# Autodesk Inventor assembly: LR_07
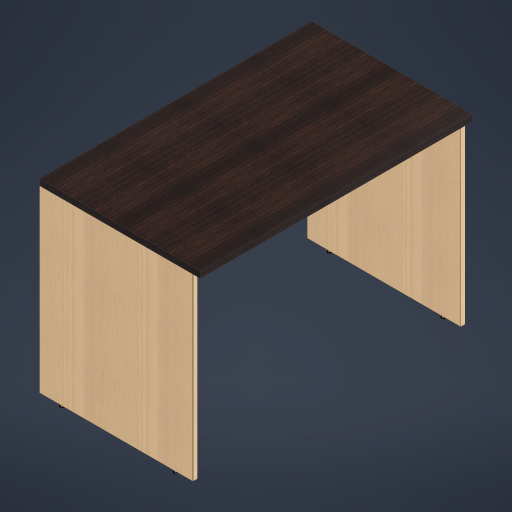
[picture p0: Inventor's stored thumbnail of the model, 512x512]
Saved by Autodesk Inventor 2024.3 (Build 283343000, 343)
## iProperties
Created: 2013-04-03
Part Number: LR_07
Document SubType Name: Assembly
Designer: User
Description: Table
Author: User
## Documents named in this file (10)
- C:\W4INV 2024 Design\PROJECTS\Living Room\Table\LR_07.iam
- C:\W4INV 2024 Design\PROJECTS\Samples\Living Room\Table\LR_0703.ipt
- C:\W4INV 2024 Design\PROJECTS\Samples\Living Room\Table\LR_0701.ipt
- C:\W4INV 2024 Design\PROJECTS\Samples\Living Room\Table\LR_0700.ipt
- C:\W4INV 2024 Design\PROJECTS\Samples\Living Room\Table\LR_0702.ipt
- C:\W4INV 2024 Design\_LIBRARY\Fixed joints\Minifix joint\MINIFIX D15 v2\Minifix D15 & Dowel L34 & Cap D15 PB T18 LH.ipt
- C:\W4INV 2024 Design\_LIBRARY\Fixed joints\Minifix joint\MINIFIX D15 v2\Minifix D15 & Dowel L34 & Cap D15 PB T18 RH.ipt
- C:\W4INV 2024 Design\_LIBRARY\Supports and legs\Supports\ADJUSTABLE SUPPORT\Support M6 H27 D18 with Bushing SB T18.ipt
- C:\W4INV 2023 Design\LIBRARY\Supports and legs\Supports\ADJUSTABLE SUPPORT.ipt
- C:\W4INV 2023 Design\LIBRARY\Fixed joints\Minifix joint\MINIFIX D15 v2.ipt
## Components (16 placed, 7 different names)
1. LR_0703-Desktop:1 — Mate:18, Mate:20, Mate:22, Mate:24
2. LR_0701-Left Leg:1 — Flush:1, Flush:2, Flush:25, Mate:10, Mate:12, Flush:27, Mate:14, Mate:16, Flush:29, Flush:31, Mate:26, Mate:30
3. LR_0700-Right Leg:1 — Flush:26, Flush:28, Flush:30, Flush:32, Mate:28, Mate:32
4. LR_0702-Support:1 — Flush:7, Flush:8, Flush:33, Flush:34, Flush:35, Flush:36
5. Support M6 H27 D18 with Bushing SB T18:5 — Mate:9, Flush:25, Mate:10
6. Support M6 H27 D18 with Bushing SB T18:6 — Mate:11, Flush:26, Mate:12
7. Support M6 H27 D18 with Bushing SB T18:7 — Mate:13, Flush:27, Mate:14
8. Support M6 H27 D18 with Bushing SB T18:8 — Mate:15, Flush:28, Mate:16
9. Minifix D15 & Dowel L34 & Cap D15 PB T18 LH:1 — Mate:17, Flush:29, Mate:18
10. Minifix D15 & Dowel L34 & Cap D15 PB T18 RH:2 — Mate:19, Flush:30, Mate:20
11. Minifix D15 & Dowel L34 & Cap D15 PB T18 RH:3 — Mate:21, Flush:31, Mate:22
12. Minifix D15 & Dowel L34 & Cap D15 PB T18 LH:4 — Mate:23, Flush:32, Mate:24
13. Minifix D15 & Dowel L34 & Cap D15 PB T18 LH:5 — Mate:25, Mate:26, Flush:33
14. Minifix D15 & Dowel L34 & Cap D15 PB T18 RH:6 — Mate:27, Mate:28, Flush:34
15. Minifix D15 & Dowel L34 & Cap D15 PB T18 RH:7 — Mate:29, Mate:30, Flush:35
16. Minifix D15 & Dowel L34 & Cap D15 PB T18 LH:8 — Mate:31, Mate:32, Flush:36
## Relationships (40: Mate 24, Flush 16)
- Flush:1 (-80 mm): LR_0701-Left Leg:1
- Flush:2 (-80 mm): LR_0701-Left Leg:1
- Flush:7 (-60 mm): LR_0702-Support:1
- Flush:8 (-60 mm): LR_0702-Support:1
- Mate:9: Support M6 H27 D18 with Bushing SB T18:5
- Flush:25 (9 mm): LR_0701-Left Leg:1 ↔ Support M6 H27 D18 with Bushing SB T18:5
- Mate:10 (17.5 mm): LR_0701-Left Leg:1 ↔ Support M6 H27 D18 with Bushing SB T18:5
- Mate:11: Support M6 H27 D18 with Bushing SB T18:6
- Flush:26 (9 mm): LR_0700-Right Leg:1 ↔ Support M6 H27 D18 with Bushing SB T18:6
- Mate:12 (17.5 mm): LR_0701-Left Leg:1 ↔ Support M6 H27 D18 with Bushing SB T18:6
- Mate:13: Support M6 H27 D18 with Bushing SB T18:7
- Flush:27 (9 mm): LR_0701-Left Leg:1 ↔ Support M6 H27 D18 with Bushing SB T18:7
- Mate:14 (17.5 mm): LR_0701-Left Leg:1 ↔ Support M6 H27 D18 with Bushing SB T18:7
- Mate:15: Support M6 H27 D18 with Bushing SB T18:8
- Flush:28 (9 mm): LR_0700-Right Leg:1 ↔ Support M6 H27 D18 with Bushing SB T18:8
- Mate:16 (17.5 mm): LR_0701-Left Leg:1 ↔ Support M6 H27 D18 with Bushing SB T18:8
- Mate:17: Minifix D15 & Dowel L34 & Cap D15 PB T18 LH:1
- Flush:29 (18 mm): LR_0701-Left Leg:1 ↔ Minifix D15 & Dowel L34 & Cap D15 PB T18 LH:1
- Mate:18: LR_0703-Desktop:1 ↔ Minifix D15 & Dowel L34 & Cap D15 PB T18 LH:1
- Mate:19: Minifix D15 & Dowel L34 & Cap D15 PB T18 RH:2
- Flush:30 (18 mm): LR_0700-Right Leg:1 ↔ Minifix D15 & Dowel L34 & Cap D15 PB T18 RH:2
- Mate:20: LR_0703-Desktop:1 ↔ Minifix D15 & Dowel L34 & Cap D15 PB T18 RH:2
- Mate:21: Minifix D15 & Dowel L34 & Cap D15 PB T18 RH:3
- Flush:31 (18 mm): LR_0701-Left Leg:1 ↔ Minifix D15 & Dowel L34 & Cap D15 PB T18 RH:3
- Mate:22: LR_0703-Desktop:1 ↔ Minifix D15 & Dowel L34 & Cap D15 PB T18 RH:3
- Mate:23: Minifix D15 & Dowel L34 & Cap D15 PB T18 LH:4
- Flush:32 (18 mm): LR_0700-Right Leg:1 ↔ Minifix D15 & Dowel L34 & Cap D15 PB T18 LH:4
- Mate:24: LR_0703-Desktop:1 ↔ Minifix D15 & Dowel L34 & Cap D15 PB T18 LH:4
- Mate:25: Minifix D15 & Dowel L34 & Cap D15 PB T18 LH:5
- Mate:26: LR_0701-Left Leg:1 ↔ Minifix D15 & Dowel L34 & Cap D15 PB T18 LH:5
- Flush:33 (18 mm): LR_0702-Support:1 ↔ Minifix D15 & Dowel L34 & Cap D15 PB T18 LH:5
- Mate:27: Minifix D15 & Dowel L34 & Cap D15 PB T18 RH:6
- Mate:28: LR_0700-Right Leg:1 ↔ Minifix D15 & Dowel L34 & Cap D15 PB T18 RH:6
- Flush:34 (18 mm): LR_0702-Support:1 ↔ Minifix D15 & Dowel L34 & Cap D15 PB T18 RH:6
- Mate:29: Minifix D15 & Dowel L34 & Cap D15 PB T18 RH:7
- Mate:30: LR_0701-Left Leg:1 ↔ Minifix D15 & Dowel L34 & Cap D15 PB T18 RH:7
- Flush:35 (18 mm): LR_0702-Support:1 ↔ Minifix D15 & Dowel L34 & Cap D15 PB T18 RH:7
- Mate:31: Minifix D15 & Dowel L34 & Cap D15 PB T18 LH:8
- Mate:32: LR_0700-Right Leg:1 ↔ Minifix D15 & Dowel L34 & Cap D15 PB T18 LH:8
- Flush:36 (18 mm): LR_0702-Support:1 ↔ Minifix D15 & Dowel L34 & Cap D15 PB T18 LH:8
